# Autodesk Inventor assembly: !gearbox_mirrored
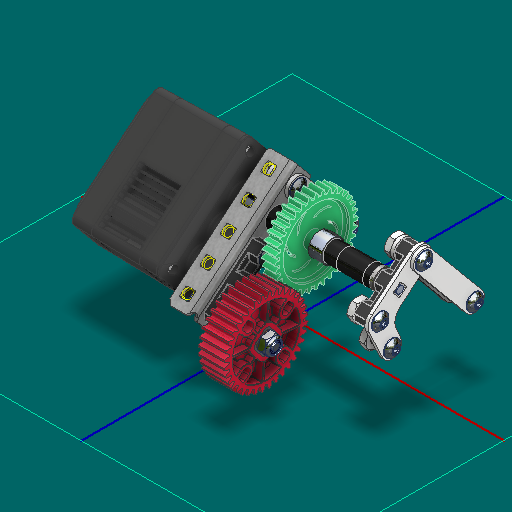
[picture p0: Inventor's stored thumbnail of the model, 512x512]
Saved by Autodesk Inventor 2025 (Build 290162000, 162)
## iProperties
Created: 2024-08-16
Part Number: !gearbox_mirrored
Document SubType Name: Assembly
Designer: averey
Author: averey
## Documents named in this file (5)
- C:\Users\avere\vex_robotics_high_stakes\hardware\cad\ATLAS\chassis\drive_pod\back_left\gearbox\!gearbox_mirrored.iam
- C:\Users\avere\vex_robotics_high_stakes\hardware\cad\ATLAS\chassis\drive_pod\back_left\gearbox\structure_mirrored.iam
- C:\Users\avere\vex_robotics_high_stakes\hardware\cad\ATLAS\chassis\drive_pod\back_left\gearbox\top_shaft_mirrored.iam
- C:\Users\avere\vex_robotics_high_stakes\hardware\cad\ATLAS\chassis\drive_pod\back_left\gearbox\V5 Motor (5.5W)_mirrored.ipt
- C:\Users\avere\vex_robotics_high_stakes\hardware\cad\ATLAS\chassis\drive_pod\back_left\gearbox\idler_screw_join_mirrored.iam
## Components (4 placed, 4 different names)
1. structure_mirrored:1 [sub-assembly] — Insert:4, Mate:1, Insert:2, Mate:2, Insert:3
2. top_shaft_mirrored:1 [sub-assembly] — Insert:4, Angle:1
3. V5 Motor (5.5W)_mirrored:1 — Angle:1, Mate:1, Insert:2
4. idler_screw_join_mirrored:1 [sub-assembly] — Mate:2, Insert:3
## Relationships (6: Insert 3, Mate 2, Angle 1)
- Insert:4 (1.27 mm): structure_mirrored:1 ↔ top_shaft_mirrored:1
- Angle:1 (0 deg): top_shaft_mirrored:1 ↔ V5 Motor (5.5W)_mirrored:1
- Mate:1: structure_mirrored:1 ↔ V5 Motor (5.5W)_mirrored:1
- Insert:2: structure_mirrored:1 ↔ V5 Motor (5.5W)_mirrored:1
- Mate:2: structure_mirrored:1 ↔ idler_screw_join_mirrored:1
- Insert:3: structure_mirrored:1 ↔ idler_screw_join_mirrored:1
